# Autodesk Inventor assembly: Arm
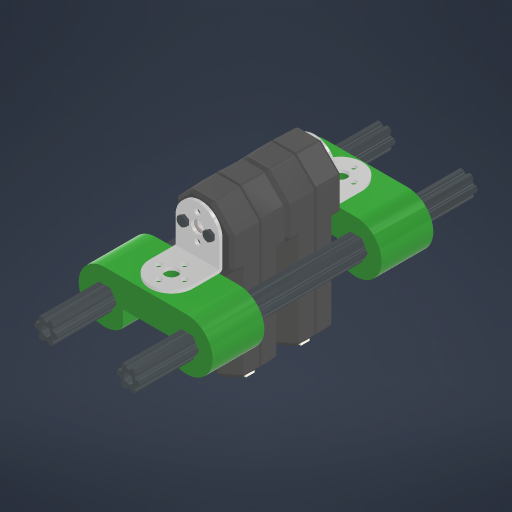
[picture p0: Inventor's stored thumbnail of the model, 512x512]
Saved by Autodesk Inventor 2024.2 (Build 282272000, 272)
## iProperties
Created: 2024-01-12
Part Number: Arm
Document SubType Name: Assembly
Designer: Allan Niles
Author: Allan Niles
## Documents named in this file (6)
- C:\Users\alniles07\Documents\Github\8400_2024_CAD\Arm.iam
- C:\Users\alniles07\Documents\Github\8400_2024_CAD\Churro Arm Mount.ipt
- C:\Users\alniles07\Documents\Github\8400_2024_CAD\Middle Churo.ipt
- C:\Users\alniles07\Documents\Github\8400_2024_CAD\Core Hex Motor.ipt
- C:\Users\alniles07\Documents\Github\8400_2024_CAD\Small Bracet.ipt
- C:\Users\alniles07\Documents\Github\8400_2024_CAD\Small Hex Screw.ipt
## Components (12 placed, 5 different names)
1. Churro Arm Mount:1 — Mate:1, Mate:2, Mate:3, Mate:4, Flush:1, Mate:9, Mate:10, Mate:13, Mate:37, Mate:38, Mate:39
2. Churro Arm Mount:2 — Mate:5, Mate:6, Flush:2, Mate:11, Mate:12, Mate:14
3. Middle Churo:1 — Mate:1, Mate:2, Flush:2
4. Middle Churo:2 — Mate:3, Mate:4, Mate:5, Mate:6, Flush:1
5. Core Hex Motor:1 — Mate:7, Mate:8, Mate:15, Mate:16, Mate:17, Mate:33, Mate:35
6. Core Hex Motor:2 — Mate:7, Mate:8, Mate:18, Mate:19, Mate:20, Mate:29, Mate:31
7. Small Bracet:1 — Mate:9, Mate:10, Mate:13, Mate:18, Mate:19, Mate:20, Mate:30, Mate:32
8. Small Bracet:2 — Mate:11, Mate:12, Mate:14, Mate:15, Mate:16, Mate:17, Mate:34, Mate:36
9. Small Hex Screw:1 — Mate:29, Mate:30
10. Small Hex Screw:2 — Mate:31, Mate:32
11. Small Hex Screw:3 — Mate:33, Mate:34
12. Small Hex Screw:4 — Mate:35, Mate:36
## Relationships (33: Mate 31, Flush 2)
- Mate:1: Churro Arm Mount:1 ↔ Middle Churo:1
- Mate:2: Churro Arm Mount:1 ↔ Middle Churo:1
- Mate:3: Churro Arm Mount:1 ↔ Middle Churo:2
- Mate:4: Churro Arm Mount:1 ↔ Middle Churo:2
- Mate:5: Churro Arm Mount:2 ↔ Middle Churo:2
- Mate:6: Churro Arm Mount:2 ↔ Middle Churo:2
- Mate:7: Core Hex Motor:1 ↔ Core Hex Motor:2
- Mate:8: Core Hex Motor:1 ↔ Core Hex Motor:2
- Flush:1 (-36.3093 mm): Churro Arm Mount:1 ↔ Middle Churo:2
- Flush:2 (36.3093 mm): Churro Arm Mount:2 ↔ Middle Churo:1
- Mate:9: Churro Arm Mount:1 ↔ Small Bracet:1
- Mate:10: Churro Arm Mount:1 ↔ Small Bracet:1
- Mate:11: Churro Arm Mount:2 ↔ Small Bracet:2
- Mate:12: Churro Arm Mount:2 ↔ Small Bracet:2
- Mate:13: Churro Arm Mount:1 ↔ Small Bracet:1
- Mate:14: Churro Arm Mount:2 ↔ Small Bracet:2
- Mate:15: Core Hex Motor:1 ↔ Small Bracet:2
- Mate:16: Core Hex Motor:1 ↔ Small Bracet:2
- Mate:17: Core Hex Motor:1 ↔ Small Bracet:2
- Mate:18: Core Hex Motor:2 ↔ Small Bracet:1
- Mate:19: Core Hex Motor:2 ↔ Small Bracet:1
- Mate:20: Core Hex Motor:2 ↔ Small Bracet:1
- Mate:29: Core Hex Motor:2 ↔ Small Hex Screw:1
- Mate:30: Small Bracet:1 ↔ Small Hex Screw:1
- Mate:31: Core Hex Motor:2 ↔ Small Hex Screw:2
- Mate:32: Small Bracet:1 ↔ Small Hex Screw:2
- Mate:33: Core Hex Motor:1 ↔ Small Hex Screw:3
- Mate:34: Small Bracet:2 ↔ Small Hex Screw:3
- Mate:35: Core Hex Motor:1 ↔ Small Hex Screw:4
- Mate:36: Small Bracet:2 ↔ Small Hex Screw:4
- Mate:37: Churro Arm Mount:1
- Mate:38: Churro Arm Mount:1
- Mate:39: Churro Arm Mount:1
